# Autodesk Inventor assembly: Full_Manual_Robot_Assembly_V4_5.11.25
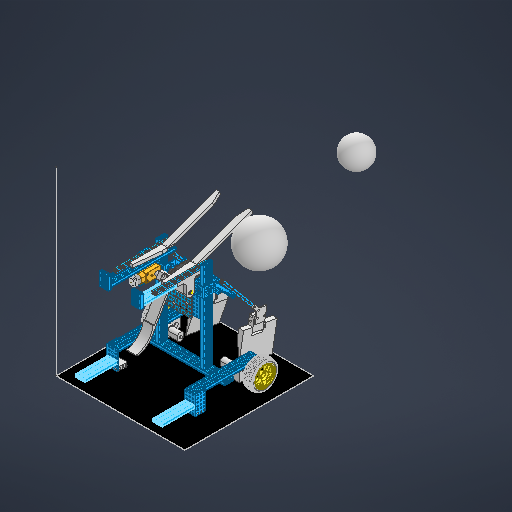
[picture p0: Inventor's stored thumbnail of the model, 512x512]
Saved by Autodesk Inventor 2026.1 (Build 301233020, 233B)
## iProperties
Created: 2025-10-16
Part Number: Full_Manual_Robot_Assembly_V4_5.11.25
Document SubType Name: Assembly
Designer: Asus
Author: Asus
## Documents named in this file (31)
- D:\KMITL\Computer_Programming\ComPro_Project\Robot_design_CAD_files\Full_Manual_Robot_Assembly_V4_5.11.25.iam
- D:\KMITL\Computer_Programming\ComPro_Project\Material_Parts_CAD_files\Metal_parts\Beam0824-224.ipt
- D:\KMITL\Computer_Programming\ComPro_Project\Field_materials_CAD_files\Manual_Robot_Size_Base.ipt
- D:\KMITL\Computer_Programming\ComPro_Project\Field_materials_CAD_files\Objective_70mm_Ball_Manual.ipt
- D:\KMITL\Computer_Programming\ComPro_Project\Field_materials_CAD_files\Objective_100mm_Ball_Manual.ipt
- D:\KMITL\Computer_Programming\ComPro_Project\Material_Parts_CAD_files\Metal_parts\Beam9x8x1-136.ipt
- D:\KMITL\Computer_Programming\ComPro_Project\Material_Parts_CAD_files\Metal_parts\Beam0824-160.ipt
- D:\KMITL\Computer_Programming\ComPro_Project\Material_Parts_CAD_files\MakeX_parts\Encoder Motor.ipt
- D:\KMITL\Computer_Programming\ComPro_Project\Material_Parts_CAD_files\Arudino_parts\Wheel D65x25.ipt
- D:\KMITL\Computer_Programming\ComPro_Project\Material_Parts_CAD_files\Metal_parts\U-Shape_Bracket.ipt
- D:\KMITL\Computer_Programming\ComPro_Project\Material_Parts_CAD_files\Electronic_parts\MEDS15 - Servo Motor.ipt
- D:\KMITL\Computer_Programming\ComPro_Project\Material_Parts_CAD_files\Metal_parts\Bracket 3x3.ipt
- D:\KMITL\Computer_Programming\ComPro_Project\Material_Parts_CAD_files\Metal_parts\Plate0324-072 V1.0.ipt
- D:\KMITL\Computer_Programming\ComPro_Project\Material_Parts_CAD_files\Metal_parts\Beam0824-032.ipt
- D:\KMITL\Computer_Programming\ComPro_Project\Field_materials_CAD_files\Manual_Robot_Height_Limit.ipt
- D:\KMITL\Computer_Programming\ComPro_Project\Material_Parts_CAD_files\Metal_parts\Bracket 3x6.ipt
- D:\KMITL\Computer_Programming\ComPro_Project\Material_Parts_CAD_files\Electronic_parts\MS-1.5A Servo.ipt
- D:\KMITL\Computer_Programming\ComPro_Project\3D_Printing_Parts_CAD_files\hand_right_1.ipt
- D:\KMITL\Computer_Programming\ComPro_Project\3D_Printing_Parts_CAD_files\hand_left_1.ipt
- D:\KMITL\Computer_Programming\ComPro_Project\Material_Parts_CAD_files\Metal_parts\Beam0824-5.ipt
- D:\KMITL\Computer_Programming\ComPro_Project\Material_Parts_CAD_files\Metal_parts\Plate 7x9.ipt
- D:\KMITL\Computer_Programming\ComPro_Project\3D_Printing_Parts_CAD_files\base_support.ipt
- D:\KMITL\Computer_Programming\ComPro_Project\Material_Parts_CAD_files\Electronic_parts\One side TT Motor v1.ipt
- D:\KMITL\Computer_Programming\ComPro_Project\3D_Printing_Parts_CAD_files\Launcher_shaft.ipt
- D:\KMITL\Computer_Programming\ComPro_Project\Material_Parts_CAD_files\MakeX_parts\Flange Bearing 4x8x3mm.ipt
- D:\KMITL\Computer_Programming\ComPro_Project\3D_Printing_Parts_CAD_files\Launcher_support.ipt
- D:\KMITL\Computer_Programming\ComPro_Project\3D_Printing_Parts_CAD_files\Launcher_Arm_V2.ipt
- D:\KMITL\Computer_Programming\ComPro_Project\3D_Printing_Parts_CAD_files\intake arm left.ipt
- D:\KMITL\Computer_Programming\ComPro_Project\3D_Printing_Parts_CAD_files\intake arm right.ipt
- D:\KMITL\Computer_Programming\ComPro_Project\3D_Printing_Parts_CAD_files\lifter arm mount.ipt
- D:\KMITL\Computer_Programming\ComPro_Project\3D_Printing_Parts_CAD_files\digital servo cap.ipt
## Components (59 placed, 30 different names)
1. Beam0824-224:3 — Rigid:4, Rigid:5, Rigid:8, Rigid:10
2. Beam0824-224:4 — Rigid:8, Rigid:11, Rigid:33, Rigid:44
3. Manual_Robot_Size_Base:1 — Flush:3, Tangent:3, Tangent:4, Mate:1, Rigid:22, Flush:5
4. Objective_70mm_Ball_Manual:1 — Tangent:1
5. Objective_100mm_Ball_Manual:1 — Tangent:2
6. Beam9x8x1-136:1 — Rigid:39, Rigid:57
7. Objective_100mm_Ball_Manual:2 — Tangent:3
8. Objective_70mm_Ball_Manual:2 — Tangent:4
9. Objective_100mm_Ball_Manual:3
10. Objective_70mm_Ball_Manual:3
11. Beam0824-160:1 — Rigid:4, Rigid:6, Rigid:23
12. Beam0824-160:2 — Rigid:5, Rigid:7, Rigid:30
13. Encoder Motor:1 — Rigid:7, Rotational:2
14. Encoder Motor:2 — Rigid:6, Rotational:1, Mate:1
15. Wheel D65x25:1 — Rotational:2
16. Wheel D65x25:2 — Rotational:1
17. U-Shape_Bracket:1 — Rigid:11, Rigid:13
18. U-Shape_Bracket:2 — Rigid:12
19. MEDS15 - Servo Motor:1 — Rigid:13, Rotational:3
20. Beam0824-224:5 — Rigid:10, Rigid:12, Rigid:34
21. Bracket 3x3:1 — Rigid:14, Rigid:61
22. Bracket 3x3:2 — Rigid:15, Rotational:3
23. Plate0324-072 V1.0:1 — Rigid:14, Rigid:15, Rigid:24, Rigid:25
24. Beam9x8x1-136:3 — Rigid:38, Rigid:59
25. Manual_Robot_Height_Limit:1 — Rigid:22
26. Bracket 3x6:1 — Rigid:30, Rigid:37, Rigid:46
27. Bracket 3x6:2 — Rigid:23, Rigid:36, Rigid:47
28. Bracket 3x3:3 — Rigid:24, Rigid:27
29. Bracket 3x3:4 — Rigid:25, Rigid:26
30. Beam0824-032:1 — Rigid:27, Rigid:39
31. Beam0824-032:2 — Rigid:26, Rigid:38
32. MS-1.5A Servo:1 — Rotational:4, Rigid:58
33. MS-1.5A Servo:2 — Rotational:5, Rigid:60
34. hand_right_1:1 — Rotational:4
35. hand_left_1:1 — Rotational:5
36. Beam9x8x1-136:4 — Rigid:33, Mate:3, Flush:4, Rigid:49, Rigid:56
37. Beam9x8x1-136:5 — Rigid:34, Rigid:40, Rigid:48, Rigid:55
38. base_support:1 — Rigid:37
39. base_support:2 — Rigid:36
40. Plate0324-072 V1.0:2 — Rigid:40, Mate:2
41. One side TT Motor v1:1 — Mate:2, Rotational:7
42. Launcher_shaft:1 — Rotational:7, Rotational:8, Rigid:52
43. Flange Bearing 4x8x3mm:1 — Rotational:8, Rotational:9
44. Flange Bearing 4x8x3mm:2 — Rotational:9, Tangent:5
45. Launcher_support:2 — Mate:3, Tangent:5, Flush:4
46. Bracket 3x6:3 — Rigid:44, Rigid:45
47. Plate 7x9:3 — Rigid:45
48. Beam0824-5:2 — Rigid:46
49. Beam0824-5:3 — Rigid:47, Flush:5
50. Beam0824-160:3 — Rigid:48, Rigid:50
51. Beam0824-5:4 — Rigid:49, Rigid:51
52. Beam0824-032:3 — Rigid:51
53. Beam0824-032:4 — Rigid:50
54. Launcher_Arm_V2:1 — Rigid:52
55. intake arm left:1 — Rigid:55
56. intake arm right:1 — Rigid:56
57. lifter arm mount:1 — Rigid:57, Rigid:58
58. lifter arm mount:2 — Rigid:59, Rigid:60
59. digital servo cap:1 — Rigid:61
## Relationships (62: WeldJoint 41, RevoluteJoint 8, Flush 5, Tangent 5, Mate 3)
- Flush:1 (-320 mm)
- Flush:2 (-320 mm)
- Flush:3 (136 mm): Manual_Robot_Size_Base:1
- Tangent:1: Objective_70mm_Ball_Manual:1
- Tangent:2: Objective_100mm_Ball_Manual:1
- Tangent:3: Manual_Robot_Size_Base:1 ↔ Objective_100mm_Ball_Manual:2
- Tangent:4: Manual_Robot_Size_Base:1 ↔ Objective_70mm_Ball_Manual:2
- Rigid:4 [WeldJoint]: Beam0824-224:3 ↔ Beam0824-160:1
- Rigid:5 [WeldJoint]: Beam0824-224:3 ↔ Beam0824-160:2
- Rigid:6 [WeldJoint]: Beam0824-160:1 ↔ Encoder Motor:2
- Rigid:7 [WeldJoint]: Beam0824-160:2 ↔ Encoder Motor:1
- Rotational:1 [RevoluteJoint]: Encoder Motor:2 ↔ Wheel D65x25:2
- Rotational:2 [RevoluteJoint]: Encoder Motor:1 ↔ Wheel D65x25:1
- Mate:1 (20.5 mm): Manual_Robot_Size_Base:1 ↔ Encoder Motor:2
- Rigid:8 [WeldJoint]: Beam0824-224:3 ↔ Beam0824-224:4
- Rigid:10 [WeldJoint]: Beam0824-224:3 ↔ Beam0824-224:5
- Rigid:11 [WeldJoint]: Beam0824-224:4 ↔ U-Shape_Bracket:1
- Rigid:12 [WeldJoint]: U-Shape_Bracket:2 ↔ Beam0824-224:5
- Rigid:13 [WeldJoint] (-7.9 mm): U-Shape_Bracket:1 ↔ MEDS15 - Servo Motor:1
- Rigid:14 [WeldJoint]: Bracket 3x3:1 ↔ Plate0324-072 V1.0:1
- Rigid:15 [WeldJoint]: Bracket 3x3:2 ↔ Plate0324-072 V1.0:1
- Rigid:22 [WeldJoint]: Manual_Robot_Size_Base:1 ↔ Manual_Robot_Height_Limit:1
- Rigid:23 [WeldJoint]: Beam0824-160:1 ↔ Bracket 3x6:2
- Rigid:24 [WeldJoint]: Plate0324-072 V1.0:1 ↔ Bracket 3x3:3
- Rigid:25 [WeldJoint]: Plate0324-072 V1.0:1 ↔ Bracket 3x3:4
- Rigid:26 [WeldJoint]: Bracket 3x3:4 ↔ Beam0824-032:2
- Rigid:27 [WeldJoint]: Bracket 3x3:3 ↔ Beam0824-032:1
- Rotational:3 [RevoluteJoint] (1.9 mm): MEDS15 - Servo Motor:1 ↔ Bracket 3x3:2
- Rigid:30 [WeldJoint]: Beam0824-160:2 ↔ Bracket 3x6:1
- Rotational:4 [RevoluteJoint]: MS-1.5A Servo:1 ↔ hand_right_1:1
- Rotational:5 [RevoluteJoint]: MS-1.5A Servo:2 ↔ hand_left_1:1
- Rigid:33 [WeldJoint]: Beam0824-224:4 ↔ Beam9x8x1-136:4
- Rigid:34 [WeldJoint]: Beam0824-224:5 ↔ Beam9x8x1-136:5
- Rigid:36 [WeldJoint]: Bracket 3x6:2 ↔ base_support:2
- Rigid:37 [WeldJoint]: Bracket 3x6:1 ↔ base_support:1
- Rigid:38 [WeldJoint]: Beam9x8x1-136:3 ↔ Beam0824-032:2
- Rigid:39 [WeldJoint]: Beam9x8x1-136:1 ↔ Beam0824-032:1
- Rigid:40 [WeldJoint]: Beam9x8x1-136:5 ↔ Plate0324-072 V1.0:2
- Mate:2: Plate0324-072 V1.0:2 ↔ One side TT Motor v1:1
- Rotational:7 [RevoluteJoint] (0.6 mm): One side TT Motor v1:1 ↔ Launcher_shaft:1
- Rotational:8 [RevoluteJoint]: Launcher_shaft:1 ↔ Flange Bearing 4x8x3mm:1
- Rotational:9 [RevoluteJoint] (8 mm): Flange Bearing 4x8x3mm:1 ↔ Flange Bearing 4x8x3mm:2
- Mate:3: Beam9x8x1-136:4 ↔ Launcher_support:2
- Tangent:5: Flange Bearing 4x8x3mm:2 ↔ Launcher_support:2
- Flush:4: Beam9x8x1-136:4 ↔ Launcher_support:2
- Rigid:44 [WeldJoint]: Beam0824-224:4 ↔ Bracket 3x6:3
- Rigid:45 [WeldJoint]: Bracket 3x6:3 ↔ Plate 7x9:3
- Rigid:46 [WeldJoint]: Bracket 3x6:1 ↔ Beam0824-5:2
- Rigid:47 [WeldJoint]: Bracket 3x6:2 ↔ Beam0824-5:3
- Rigid:48 [WeldJoint]: Beam9x8x1-136:5 ↔ Beam0824-160:3
- Rigid:49 [WeldJoint]: Beam9x8x1-136:4 ↔ Beam0824-5:4
- Rigid:50 [WeldJoint]: Beam0824-160:3 ↔ Beam0824-032:4
- Rigid:51 [WeldJoint]: Beam0824-5:4 ↔ Beam0824-032:3
- Rigid:52 [WeldJoint]: Launcher_shaft:1 ↔ Launcher_Arm_V2:1
- Flush:5: Manual_Robot_Size_Base:1 ↔ Beam0824-5:3
- Rigid:55 [WeldJoint]: Beam9x8x1-136:5 ↔ intake arm left:1
- Rigid:56 [WeldJoint]: Beam9x8x1-136:4 ↔ intake arm right:1
- Rigid:57 [WeldJoint]: Beam9x8x1-136:1 ↔ lifter arm mount:1
- Rigid:58 [WeldJoint]: MS-1.5A Servo:1 ↔ lifter arm mount:1
- Rigid:59 [WeldJoint]: Beam9x8x1-136:3 ↔ lifter arm mount:2
- Rigid:60 [WeldJoint]: MS-1.5A Servo:2 ↔ lifter arm mount:2
- Rigid:61 [WeldJoint]: Bracket 3x3:1 ↔ digital servo cap:1
